# Autodesk Inventor assembly: Assembly1
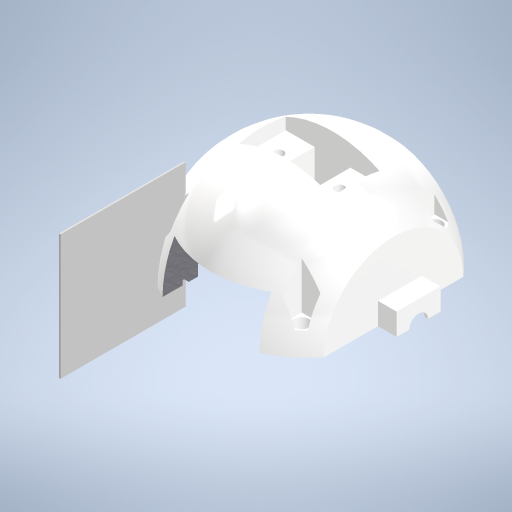
[picture p0: Inventor's stored thumbnail of the model, 512x512]
Saved by Autodesk Inventor 2023 (Build 270158000, 158)
## iProperties
Created: 2022-10-24
Part Number: Assembly1
Document SubType Name: Assembly
Designer: ellie
Author: ellie
## Documents named in this file (5)
- C:\Users\ellie\Documents\github\tanekonsat2022_runback\machinary\assenbly\Assembly1.iam
- C:\Users\ellie\Documents\github\tanekonsat2022_runback\machinary\body\body back.ipt
- C:\Users\ellie\Documents\github\tanekonsat2022_runback\machinary\body\body back for main 3.ipt
- C:\Users\ellie\Documents\github\tanekonsat2022_runback\machinary\body\body front.ipt
- C:\Users\ellie\Documents\github\tanekonsat2022_runback\machinary\parts\almi1.ipt
## Components (5 placed, 3 different names)
1. body back:1 — メイト:1, メイト:2, メイト:3, メイト:4, メイト:5, メイト:6
2. body back:2 — メイト:1, メイト:2, メイト:3
3. body back:3 — メイト:4, メイト:5, メイト:6
4. base front:1 — メイト:7
5. almi1:1 — メイト:7
## Relationships (7: Mate 7)
- メイト:1 [Mate]: body back:1 ↔ body back:2
- メイト:2 [Mate]: body back:1 ↔ body back:2
- メイト:3 [Mate]: body back:1 ↔ body back:2
- メイト:4 [Mate]: body back:1 ↔ body back:3
- メイト:5 [Mate]: body back:1 ↔ body back:3
- メイト:6 [Mate]: body back:1 ↔ body back:3
- メイト:7 [Mate]: base front:1 ↔ almi1:1
